# Autodesk Inventor assembly: Odom Rail
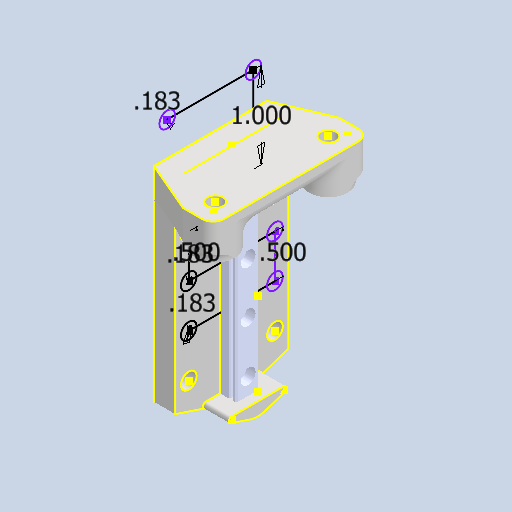
[picture p0: Inventor's stored thumbnail of the model, 512x512]
Saved by Autodesk Inventor 2025.1 (Build 291241020, 241B)
## iProperties
Created: 2024-12-18
Part Number: Odom Rail
Document SubType Name: Assembly
Designer: Juan
Author: Juan
## Documents named in this file (3)
- C:\Users\AtuStem\Documents\GitHub\ATUM-V5RC-High-Stakes-CAD\Robot\Subassemblies\Odom Rail.iam
- C:\Users\AtuStem\Documents\GitHub\ATUM-V5RC-High-Stakes-CAD\Odometers_Collin\Linear_Mount_3BY.ipt
- C:\Users\AtuStem\Documents\GitHub\ATUM-V5RC-High-Stakes-CAD\Odometers_Collin\Linear Rail Files\LinearRail-LWL7B-100mm\LinearRail-LWL7B-100mm\LinearRail-LWL7B-100mm.ipt
## Components (2 placed, 2 different names)
1. Linear_Mount_3BY:1
2. LinearRail-LWL7B-100mm:1
## Relationships (3: Mate 3)
- [Mate]: Linear_Mount_3BY:1 ↔ LinearRail-LWL7B-100mm:1
- [Mate]: Linear_Mount_3BY:1 ↔ LinearRail-LWL7B-100mm:1
- [Mate]: Linear_Mount_3BY:1 ↔ LinearRail-LWL7B-100mm:1
## Named parameters: d1946_d1905 = 0 mm, d1947_d1906 = 0 mm, d1948_d1907 = 0 mm
